# Autodesk Inventor assembly: LINEAR_INTAKE_ASSY
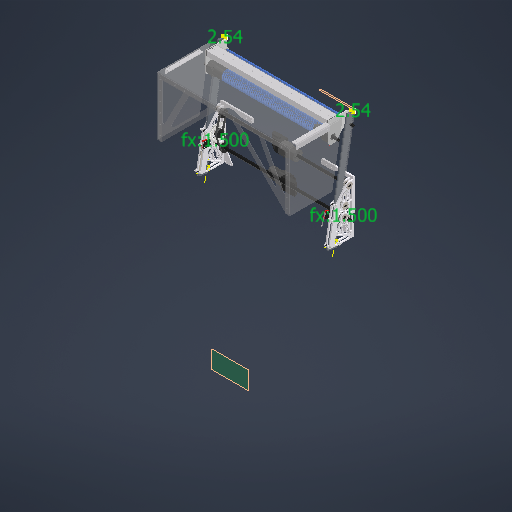
[picture p0: Inventor's stored thumbnail of the model, 512x512]
Saved by Autodesk Inventor 2026.2 (Build 302298010, 298A)
## iProperties
Created: 2026-04-01
Part Number: LINEAR_INTAKE_ASSY
Document SubType Name: Assembly
Designer: 4aida
Author: 4aida
## Documents named in this file (36)
- C:\Users\4aida\OneDrive\Documents\GitHub\2026-Robot-Mechanical\LINEAR_INTAKE\LINEAR_INTAKE_ASSY.iam
- C:\Users\4aida\OneDrive\Documents\GitHub\2026-Robot-Mechanical\LINEAR_INTAKE\0.5_Jack_Shaft.ipt
- C:\Users\4aida\OneDrive\Documents\GitHub\2026-Robot-Mechanical\#1_CAD Library\Electronics\CONTROLS,SPARK_FLEX.ipt
- C:\Users\4aida\OneDrive\Documents\GitHub\2026-Robot-Mechanical\#1_CAD Library\Motors\MOTOR,REV,NEO,VORTEX.ipt
- C:\Users\4aida\OneDrive\Documents\GitHub\2026-Robot-Mechanical\LINEAR_INTAKE\RACK_LINEARINTAKE.ipt
- C:\Users\4aida\OneDrive\Documents\GitHub\2026-Robot-Mechanical\LINEAR_INTAKE\10DP_Pinion Gear.iam
- C:\Users\4aida\OneDrive\Documents\GitHub\2026-Robot-Mechanical\#1_CAD Library\Power Transmission\Bearings\PURCHASED,HEX_BEARING.ipt
- C:\Users\4aida\OneDrive\Documents\GitHub\2026-Robot-Mechanical\LINEAR_INTAKE\INTAKE_OUTSIDE_PLATE.ipt
- C:\Users\4aida\OneDrive\Documents\GitHub\2026-Robot-Mechanical\LINEAR_INTAKE\RACK_GUIDES.ipt
- C:\Users\4aida\OneDrive\Documents\GitHub\2026-Robot-Mechanical\LINEAR_INTAKE\CAST,2inOD,ROLLER.ipt
- C:\Users\4aida\OneDrive\Documents\GitHub\2026-Robot-Mechanical\LINEAR_INTAKE\10dp_Ratio_Gears_INTAKE.iam
- C:\Users\4aida\OneDrive\Documents\GitHub\2026-Robot-Mechanical\LINEAR_INTAKE\INTAKE_EXT_PULLYS.ipt
- C:\Users\4aida\OneDrive\Documents\GitHub\2026-Robot-Mechanical\LINEAR_INTAKE\55t_Belt.ipt
- C:\Users\4aida\OneDrive\Documents\GitHub\2026-Robot-Mechanical\LINEAR_INTAKE\12mm_OD_BEARING.ipt
- C:\Users\4aida\OneDrive\Documents\GitHub\2026-Robot-Mechanical\LINEAR_INTAKE\fastenal_1140891.ipt
- C:\Users\4aida\OneDrive\Documents\GitHub\2026-Robot-Mechanical\LINEAR_INTAKE\SINGLE_BEARING_SPACER.ipt
- C:\Users\4aida\OneDrive\Documents\GitHub\2026-Robot-Mechanical\LINEAR_INTAKE\double_BEARING_SPACER.ipt
- C:\Users\4aida\OneDrive\Documents\GitHub\2026-Robot-Mechanical\LINEAR_INTAKE\INTAKE_SWERVE_MOUNT.ipt
- C:\Users\4aida\OneDrive\Documents\GitHub\2026-Robot-Mechanical\LINEAR_INTAKE\MOUTER_MOUNT_INTAKE.ipt
- C:\Users\4aida\OneDrive\Documents\GitHub\2026-Robot-Mechanical\LINEAR_INTAKE\INTAKE_INSIDE_PLATE.ipt
- C:\Users\4aida\OneDrive\Documents\GitHub\2026-Robot-Mechanical\LINEAR_INTAKE\INTAKE_BACK_MOUNT_PLATE.ipt
- C:\Users\4aida\OneDrive\Documents\GitHub\2026-Robot-Mechanical\LINEAR_INTAKE\PULLY_HEX_SHAFT_INTAKE.ipt
- C:\Users\4aida\OneDrive\Documents\GitHub\2026-Robot-Mechanical\LINEAR_INTAKE\PINION_SHAFT_INTAKE.ipt
- C:\Users\4aida\OneDrive\Documents\GitHub\2026-Robot-Mechanical\LINEAR_INTAKE\TETHLON_TAPE.ipt
- C:\Users\4aida\OneDrive\Documents\GitHub\2026-Robot-Mechanical\LINEAR_INTAKE\PINION_SPACER_INTAKE.ipt
- C:\Users\4aida\OneDrive\Documents\GitHub\2026-Robot-Mechanical\LINEAR_INTAKE\PULLY_SPACER_INTAKE.ipt
- C:\Users\4aida\OneDrive\Documents\GitHub\2026-Robot-Mechanical\LINEAR_INTAKE\1.25IN Roller.iam
- C:\Users\4aida\OneDrive\Documents\GitHub\2026-Robot-Mechanical\LINEAR_INTAKE\CRASH_BAR_INTAKE.ipt
- C:\Users\4aida\OneDrive\Documents\GitHub\2026-Robot-Mechanical\LINEAR_INTAKE\TUBE_PLUGS.ipt
- C:\Users\4aida\OneDrive\Documents\GitHub\2026-Robot-Mechanical\#1_CAD Library\Electronics\CONTROLS,LIMIT_SWITCH,VEX.iam
- C:\Users\4aida\OneDrive\Documents\GitHub\2026-Robot-Mechanical\LINEAR_INTAKE\INSIDE_INTAKE_PLATE.ipt
- C:\Users\4aida\OneDrive\Documents\GitHub\2026-Robot-Mechanical\LINEAR_INTAKE\FRONT_INTAKE_LEXAN.ipt
- C:\Users\4aida\OneDrive\Documents\GitHub\2026-Robot-Mechanical\LINEAR_INTAKE\SIDE_INTAKE_LEXAN.ipt
- C:\Users\4aida\OneDrive\Documents\GitHub\2026-Robot-Mechanical\LINEAR_INTAKE\SIDE_INTAKE_LEXAN_MIR.ipt
- C:\Users\4aida\OneDrive\Documents\GitHub\2026-Robot-Mechanical\LINEAR_INTAKE\TOP_INTAKE_LEXAN.ipt
- C:\Users\4aida\OneDrive\Documents\GitHub\2026-Robot-Mechanical\LINEAR_INTAKE\LEXAN_CORNER_MOUNT.ipt
## Components (130 placed, 35 different names)
1. 0.5_Jack_Shaft:1 — Flush:61
2. CONTROLS,SPARK_FLEX:1 — Mate:104, Angle:1, Mate:132, Mate:134
3. MOTOR,REV,NEO,VORTEX:1 — Mate:133
4. RACK_LINEARINTAKE:1 — Mate:149, Mate:230
5. 10DP_Pinion Gear:1 [sub-assembly] — Mate:19, Mate:201
6. PURCHASED,HEX_BEARING:1
7. PURCHASED,HEX_BEARING:2 — Mate:151, Flush:53, Flush:54
8. INTAKE_OUTSIDE_PLATE:1 — Mate:66, Mate:67, Insert:3, Mate:121, Mate:122, Mate:123, Mate:124, Mate:125, Mate:126, Mate:128, Mate:129, Insert:4, Insert:5, Insert:6, Insert:7, Insert:8, Insert:9, Flush:27, Flush:28, Mate:169, Flush:31, Flush:39, Mate:200, Flush:40
9. INTAKE_OUTSIDE_PLATE:2 — Flush:18, Mate:60, Mate:63, Insert:1, Mate:131, Flush:30, Insert:21, Insert:22, Insert:23, Insert:24, Insert:25, Insert:27, Mate:171, Mate:174, Flush:37, Mate:196, Mate:198, Flush:42, Mate:316, Mate:317
10. RACK_LINEARINTAKE:2
11. 10DP_Pinion Gear:2 [sub-assembly] — Mate:19, Mate:195
12. RACK_GUIDES:1 — Mate:272, Angle:5, Flush:56
13. RACK_GUIDES:4 — Flush:18, Mate:196
14. PURCHASED,HEX_BEARING:3 — Mate:60, Mate:63, Mate:194, Mate:195, Mate:203, Mate:204
15. PURCHASED,HEX_BEARING:4 — Mate:106, Mate:177, Mate:178, Mate:192
16. PURCHASED,HEX_BEARING:5 — Mate:96, Mate:154, Mate:157
17. PURCHASED,HEX_BEARING:6 — Mate:66, Mate:67, Mate:189, Flush:34, Mate:190, Mate:202
18. PURCHASED,HEX_BEARING:7 — Mate:107, Mate:115, Mate:176, Mate:179, Mate:180, Mate:185
19. PURCHASED,HEX_BEARING:8 — Mate:113, Mate:173, Mate:175, Mate:205, Mate:206
20. PURCHASED,HEX_BEARING:9 — Mate:152, Mate:153, Mate:207
21. PURCHASED,HEX_BEARING:10 — Insert:1, Mate:184
22. PURCHASED,HEX_BEARING:11 — Mate:94, Mate:95, Mate:155, Mate:156
23. PURCHASED,HEX_BEARING:12 — Insert:3, Mate:188
24. 55t_Belt:1 — Mate:110, Mate:111, Mate:112, Mate:182, Mate:306
25. 55t_Belt:2 — Mate:99, Mate:100, Mate:101, Mate:102, Mate:158, Mate:293
26. 10dp_Ratio_Gears_INTAKE:3 [sub-assembly] — Mate:94, Mate:95, Mate:96, Mate:97, Mate:98, Mate:154, Mate:191
27. INTAKE_EXT_PULLYS:5 — Mate:97, Mate:98, Mate:99, Mate:100, Flush:33, Mate:186, Mate:187
28. INTAKE_EXT_PULLYS:6 — Mate:101, Mate:102, Mate:208
29. 10dp_Ratio_Gears_INTAKE:4 [sub-assembly] — Mate:106, Mate:107, Mate:108, Mate:109, Mate:110, Flush:35, Mate:193
30. INTAKE_EXT_PULLYS:7 — Mate:108, Mate:109, Mate:111, Flush:26, Mate:115, Flush:32, Mate:183
31. INTAKE_EXT_PULLYS:9 — Mate:112, Flush:26, Mate:113
32. 12mm_OD_BEARING:1 — Mate:121, Mate:124, Insert:13
33. 12mm_OD_BEARING:2 — Mate:119, Mate:120
34. 12mm_OD_BEARING:3 — Mate:125, Insert:11
35. 12mm_OD_BEARING:4 — Mate:122, Mate:123, Insert:15
36. 12mm_OD_BEARING:5 — Mate:119, Mate:120, Insert:10
37. 12mm_OD_BEARING:6 — Mate:126, Insert:12
38. 12mm_OD_BEARING:12 — Mate:128, Mate:129, Insert:14
39. fastenal_1140891:1 — Insert:4
40. fastenal_1140891:2 — Insert:5
41. fastenal_1140891:3 — Insert:8
42. fastenal_1140891:4 — Insert:9
43. fastenal_1140891:5 — Insert:7
44. fastenal_1140891:6 — Insert:6
45. SINGLE_BEARING_SPACER:3 — Insert:10
46. double_BEARING_SPACER:1 — Insert:11
47. double_BEARING_SPACER:2 — Insert:15
48. double_BEARING_SPACER:3 — Insert:12
49. double_BEARING_SPACER:4 — Insert:13
50. double_BEARING_SPACER:5 — Insert:14
51. INTAKE_SWERVE_MOUNT:1 — Flush:27, Flush:28, Flush:29, Mate:150
52. INTAKE_SWERVE_MOUNT:2 — Mate:131, Flush:29, Flush:30, Mate:172, Mate:181, Flush:48
53. MOUTER_MOUNT_INTAKE:1 — Mate:132, Mate:133, Mate:134
54. 12mm_OD_BEARING:13 — Mate:135, Mate:136
55. fastenal_1140891:7 — Mate:135, Mate:136, Insert:24
56. double_BEARING_SPACER:6
57. 12mm_OD_BEARING:14
58. fastenal_1140891:8 — Insert:25
59. double_BEARING_SPACER:7
60. 12mm_OD_BEARING:15
61. fastenal_1140891:9 — Insert:23
62. double_BEARING_SPACER:8
63. 12mm_OD_BEARING:16
64. fastenal_1140891:10 — Insert:21
65. double_BEARING_SPACER:9
66. 12mm_OD_BEARING:17
67. fastenal_1140891:11 — Insert:22
68. double_BEARING_SPACER:10
69. 12mm_OD_BEARING:18
70. 12mm_OD_BEARING:19 — Mate:147
71. fastenal_1140891:12 — Mate:147, Mate:148, Insert:27
72. SINGLE_BEARING_SPACER:4 — Mate:148
73. INTAKE_INSIDE_PLATE:1 — Mate:149, Mate:150, Mate:151, Mate:152, Mate:153, Mate:155, Mate:156, Mate:157, Mate:158, Mate:168, Flush:38, Mate:199, Flush:41, Mate:289, Mate:290, Mate:291, Mate:292, Mate:300
74. INTAKE_BACK_MOUNT_PLATE:1 — Mate:168, Mate:169, Flush:31
75. INTAKE_BACK_MOUNT_PLATE:2 — Mate:171, Mate:315, Mate:316, Mate:317
76. INTAKE_INSIDE_PLATE:3 — Mate:172, Mate:173, Mate:174, Mate:175, Mate:176, Mate:177, Mate:178, Mate:179, Mate:180, Mate:181, Flush:36, Mate:197, Flush:43, Mate:286, Mate:287, Mate:288, Insert:28, Angle:6
77. PULLY_HEX_SHAFT_INTAKE:1 — Mate:182, Flush:32, Mate:183, Mate:184, Mate:185
78. PULLY_HEX_SHAFT_INTAKE:2 — Flush:33, Mate:186, Mate:187, Mate:188
79. PINION_SHAFT_INTAKE:1 — Mate:189, Flush:34, Mate:190, Mate:191
80. PINION_SHAFT_INTAKE:2 — Mate:192, Flush:35, Mate:193, Mate:194
81. TETHLON_TAPE:1 — Flush:36, Mate:197, Flush:43
82. TETHLON_TAPE:2 — Flush:38, Mate:198, Flush:42
83. TETHLON_TAPE:3 — Flush:37, Mate:200, Flush:40
84. TETHLON_TAPE:4 — Flush:39, Mate:199, Flush:41
85. PINION_SPACER_INTAKE:1 — Mate:203, Mate:204
86. PINION_SPACER_INTAKE:2 — Mate:201, Mate:202
87. PULLY_SPACER_INTAKE:1 — Mate:205, Mate:206
88. PULLY_SPACER_INTAKE:2 — Mate:207, Mate:208
89. CRASH_BAR_INTAKE:1 — Mate:220, Mate:224, Mate:225, Mate:226, Mate:227, Mate:228, Mate:229, Mate:230, Angle:2, Mate:274, Flush:55
90. TUBE_PLUGS:1 — Mate:227, Mate:228, Mate:229, Mate:235, Mate:236, Mate:263
91. TUBE_PLUGS:2 — Mate:224, Mate:225, Mate:226, Mate:231, Mate:232, Mate:233
92. INSIDE_INTAKE_PLATE:1 — Mate:231, Mate:232, Mate:233, Mate:242, Mate:243, Mate:244, Mate:249, Mate:250, Angle:4
93. 1.25IN Roller:6 [sub-assembly] — Mate:242, Mate:245, Mate:253, Mate:254, Flush:49
94. INSIDE_INTAKE_PLATE:2 — Mate:235, Mate:236, Mate:240, Mate:241, Angle:3, Mate:262, Mate:263
95. CONTROLS,SPARK_FLEX:4 — Mate:240, Angle:3
96. MOTOR,REV,NEO,VORTEX:4 — Mate:241
97. PURCHASED,HEX_BEARING:14 — Mate:243, Mate:244, Mate:245, Mate:271, Mate:273
98. CAST,2inOD,ROLLER:9 — Mate:251, Mate:252, Mate:264, Mate:267
99. CONTROLS,SPARK_FLEX:5 — Mate:249, Angle:4, Mate:270
100. MOTOR,REV,NEO,VORTEX:5 — Mate:250, Mate:251, Mate:252
101. 1.25IN Roller:7 [sub-assembly] — Mate:253, Mate:254, Mate:255, Mate:256, Flush:49, Flush:50, Flush:51
102. 1.25IN Roller:8 [sub-assembly] — Mate:255, Mate:256, Flush:50, Mate:257, Mate:258, Flush:51
103. 1.25IN Roller:9 [sub-assembly] — Mate:257, Mate:258, Mate:259, Mate:260, Flush:52
104. 1.25IN Roller:10 [sub-assembly] — Mate:259, Mate:260, Flush:52, Mate:261
105. PURCHASED,HEX_BEARING:15 — Mate:261, Mate:262
106. CAST,2inOD,ROLLER:10 — Mate:264, Mate:265, Mate:267, Mate:268
107. CAST,2inOD,ROLLER:11 — Mate:265, Mate:266, Mate:268, Mate:269
108. CAST,2inOD,ROLLER:12 — Mate:266, Mate:269
109. 0.5_Jack_Shaft:2 — Flush:53, Mate:270
110. 0.5_Jack_Shaft:3 — Flush:54, Mate:271
111. FRONT_INTAKE_LEXAN:2 — Mate:274, Flush:55, Flush:56, Mate:275, Mate:276, Flush:57, Mate:277, Flush:58, Mate:278, Flush:60, Mate:280, Mate:282, Mate:285
112. SIDE_INTAKE_LEXAN:1 — Mate:275, Mate:276, Flush:57, Mate:281
113. SIDE_INTAKE_LEXAN_MIR:1 — Mate:277, Flush:58, Mate:278, Mate:279, Flush:59, Mate:283, Mate:284
114. TOP_INTAKE_LEXAN:1 — Mate:279, Flush:59, Flush:60
115. LEXAN_CORNER_MOUNT:1 — Mate:280, Mate:281, Mate:285
116. LEXAN_CORNER_MOUNT:2 — Mate:282, Mate:283, Mate:284
117. CONTROLS,LIMIT_SWITCH,VEX:2 [sub-assembly] — Mate:286, Mate:287, Mate:288
118. CONTROLS,LIMIT_SWITCH,VEX:3 [sub-assembly] — Mate:289, Mate:290, Mate:291
119. PURCHASED,HEX_BEARING:16 — Mate:292, Mate:294, Mate:299, Mate:300
120. 55t_Belt:3 — Mate:293, Mate:294, Mate:295, Mate:296
121. INTAKE_EXT_PULLYS:10 — Mate:295, Mate:296, Mate:297, Mate:298, Mate:301
122. PULLY_SPACER_INTAKE:3 — Mate:297, Mate:298, Mate:299
123. 0.5_Jack_Shaft:4 — Mate:301, Flush:61
124. PURCHASED,HEX_BEARING:17 — Insert:28
125. INTAKE_EXT_PULLYS:11 — Mate:305, Mate:307, Mate:308
126. PULLY_SPACER_INTAKE:4 — Mate:305
127. 55t_Belt:4 — Mate:306, Mate:307, Mate:308
128. CONTROLS,SPARK_FLEX:6
129. MOTOR,REV,NEO,VORTEX:6
130. MOUTER_MOUNT_INTAKE:2 — Mate:315, Angle:6
## Relationships (289: Mate 212, Flush 44, Insert 27, Angle 6)
- [Mate]: CONTROLS,SPARK_FLEX:1 ↔ MOTOR,REV,NEO,VORTEX:1
- [Mate]: CONTROLS,SPARK_FLEX:1 ↔ MOTOR,REV,NEO,VORTEX:1
- [Mate]: CONTROLS,SPARK_FLEX:1 ↔ MOTOR,REV,NEO,VORTEX:1
- [Mate]: 0.5_Jack_Shaft:1 ↔ CONTROLS,SPARK_FLEX:1
- [Mate]: 0.5_Jack_Shaft:1 ↔ MOTOR,REV,NEO,VORTEX:1
- [Flush]: RACK_LINEARINTAKE:1 ↔ 10DP_Pinion Gear:1
- [Flush]: 0.5_Jack_Shaft:1 ↔ PURCHASED,HEX_BEARING:2
- [Flush]: 0.5_Jack_Shaft:1 ↔ PURCHASED,HEX_BEARING:1
- [Mate]: 0.5_Jack_Shaft:1 ↔ PURCHASED,HEX_BEARING:1
- [Mate]: 0.5_Jack_Shaft:1 ↔ PURCHASED,HEX_BEARING:2
- [Mate]: 0.5_Jack_Shaft:1 ↔ PURCHASED,HEX_BEARING:2
- [Mate]: 0.5_Jack_Shaft:1 ↔ PURCHASED,HEX_BEARING:1
- [Mate]: PURCHASED,HEX_BEARING:2 ↔ INTAKE_OUTSIDE_PLATE:1
- [Mate]: PURCHASED,HEX_BEARING:2 ↔ INTAKE_OUTSIDE_PLATE:1
- [Flush] (6 mm): RACK_LINEARINTAKE:1 ↔ INTAKE_OUTSIDE_PLATE:1
- [Mate] (5.2705 mm): RACK_LINEARINTAKE:1 ↔ INTAKE_OUTSIDE_PLATE:1
- [Mate]: PURCHASED,HEX_BEARING:1 ↔ INTAKE_OUTSIDE_PLATE:2
- [Mate]: PURCHASED,HEX_BEARING:1 ↔ INTAKE_OUTSIDE_PLATE:2
- [Flush]: RACK_LINEARINTAKE:2 ↔ 10DP_Pinion Gear:2
- [Flush]: RACK_LINEARINTAKE:1 ↔ RACK_LINEARINTAKE:2
- [Flush]: RACK_LINEARINTAKE:1 ↔ RACK_LINEARINTAKE:2
- Mate:19: 10DP_Pinion Gear:1 ↔ 10DP_Pinion Gear:2
- [Mate]: RACK_LINEARINTAKE:1 ↔ RACK_GUIDES:1
- [Mate]: RACK_LINEARINTAKE:2 ↔ RACK_GUIDES:4
- [Flush]: RACK_LINEARINTAKE:2 ↔ RACK_GUIDES:4
- [Flush]: RACK_LINEARINTAKE:2 ↔ RACK_GUIDES:4
- [Flush]: RACK_LINEARINTAKE:1 ↔ RACK_GUIDES:1
- [Flush]: RACK_LINEARINTAKE:1 ↔ RACK_GUIDES:1
- Flush:18: INTAKE_OUTSIDE_PLATE:2 ↔ RACK_GUIDES:4
- Mate:60: INTAKE_OUTSIDE_PLATE:2 ↔ PURCHASED,HEX_BEARING:3
- Mate:63: INTAKE_OUTSIDE_PLATE:2 ↔ PURCHASED,HEX_BEARING:3
- Mate:66: INTAKE_OUTSIDE_PLATE:1 ↔ PURCHASED,HEX_BEARING:6
- Mate:67: INTAKE_OUTSIDE_PLATE:1 ↔ PURCHASED,HEX_BEARING:6
- Insert:1: INTAKE_OUTSIDE_PLATE:2 ↔ PURCHASED,HEX_BEARING:10
- Insert:3: INTAKE_OUTSIDE_PLATE:1 ↔ PURCHASED,HEX_BEARING:12
- Mate:94: PURCHASED,HEX_BEARING:11 ↔ 10dp_Ratio_Gears_INTAKE:3
- Mate:95: PURCHASED,HEX_BEARING:11 ↔ 10dp_Ratio_Gears_INTAKE:3
- Mate:96: PURCHASED,HEX_BEARING:5 ↔ 10dp_Ratio_Gears_INTAKE:3
- Mate:97: 10dp_Ratio_Gears_INTAKE:3 ↔ INTAKE_EXT_PULLYS:5
- Mate:98: 10dp_Ratio_Gears_INTAKE:3 ↔ INTAKE_EXT_PULLYS:5
- Mate:99: 55t_Belt:2 ↔ INTAKE_EXT_PULLYS:5
- Mate:100: 55t_Belt:2 ↔ INTAKE_EXT_PULLYS:5
- Mate:101: 55t_Belt:2 ↔ INTAKE_EXT_PULLYS:6
- Mate:102: 55t_Belt:2 ↔ INTAKE_EXT_PULLYS:6
- Mate:104: CONTROLS,SPARK_FLEX:1
- Mate:106: PURCHASED,HEX_BEARING:4 ↔ 10dp_Ratio_Gears_INTAKE:4
- Mate:107: PURCHASED,HEX_BEARING:7 ↔ 10dp_Ratio_Gears_INTAKE:4
- Mate:108: 10dp_Ratio_Gears_INTAKE:4 ↔ INTAKE_EXT_PULLYS:7
- Mate:109: 10dp_Ratio_Gears_INTAKE:4 ↔ INTAKE_EXT_PULLYS:7
- Mate:110: 55t_Belt:1 ↔ 10dp_Ratio_Gears_INTAKE:4
- Mate:111: 55t_Belt:1 ↔ INTAKE_EXT_PULLYS:7
- Mate:112: 55t_Belt:1 ↔ INTAKE_EXT_PULLYS:9
- Flush:26: INTAKE_EXT_PULLYS:7 ↔ INTAKE_EXT_PULLYS:9
- Mate:113: PURCHASED,HEX_BEARING:8 ↔ INTAKE_EXT_PULLYS:9
- Mate:115: PURCHASED,HEX_BEARING:7 ↔ INTAKE_EXT_PULLYS:7
- Angle:1 (0 deg): CONTROLS,SPARK_FLEX:1
- Mate:119: 12mm_OD_BEARING:2 ↔ 12mm_OD_BEARING:5
- Mate:120: 12mm_OD_BEARING:2 ↔ 12mm_OD_BEARING:5
- Mate:121: INTAKE_OUTSIDE_PLATE:1 ↔ 12mm_OD_BEARING:1
- Mate:122: INTAKE_OUTSIDE_PLATE:1 ↔ 12mm_OD_BEARING:4
- Mate:123: INTAKE_OUTSIDE_PLATE:1 ↔ 12mm_OD_BEARING:4
- Mate:124: INTAKE_OUTSIDE_PLATE:1 ↔ 12mm_OD_BEARING:1
- Mate:125: INTAKE_OUTSIDE_PLATE:1 ↔ 12mm_OD_BEARING:3
- Mate:126: INTAKE_OUTSIDE_PLATE:1 ↔ 12mm_OD_BEARING:6
- Mate:128: INTAKE_OUTSIDE_PLATE:1 ↔ 12mm_OD_BEARING:12
- Mate:129: INTAKE_OUTSIDE_PLATE:1 ↔ 12mm_OD_BEARING:12
- Insert:4: INTAKE_OUTSIDE_PLATE:1 ↔ fastenal_1140891:1
- Insert:5: INTAKE_OUTSIDE_PLATE:1 ↔ fastenal_1140891:2
- Insert:6: INTAKE_OUTSIDE_PLATE:1 ↔ fastenal_1140891:6
- Insert:7: INTAKE_OUTSIDE_PLATE:1 ↔ fastenal_1140891:5
- Insert:8: INTAKE_OUTSIDE_PLATE:1 ↔ fastenal_1140891:3
- Insert:9: INTAKE_OUTSIDE_PLATE:1 ↔ fastenal_1140891:4
- Insert:10: 12mm_OD_BEARING:5 ↔ SINGLE_BEARING_SPACER:3
- Insert:11: 12mm_OD_BEARING:3 ↔ double_BEARING_SPACER:1
- Insert:12: 12mm_OD_BEARING:6 ↔ double_BEARING_SPACER:3
- Insert:13: 12mm_OD_BEARING:1 ↔ double_BEARING_SPACER:4
- Insert:14: 12mm_OD_BEARING:12 ↔ double_BEARING_SPACER:5
- Insert:15: 12mm_OD_BEARING:4 ↔ double_BEARING_SPACER:2
- Flush:27: INTAKE_OUTSIDE_PLATE:1 ↔ INTAKE_SWERVE_MOUNT:1
- Flush:28 (-12.2199 mm): INTAKE_OUTSIDE_PLATE:1 ↔ INTAKE_SWERVE_MOUNT:1
- Mate:131: INTAKE_OUTSIDE_PLATE:2 ↔ INTAKE_SWERVE_MOUNT:2
- Flush:29: INTAKE_SWERVE_MOUNT:1 ↔ INTAKE_SWERVE_MOUNT:2
- Flush:30: INTAKE_OUTSIDE_PLATE:2 ↔ INTAKE_SWERVE_MOUNT:2
- Mate:132: CONTROLS,SPARK_FLEX:1 ↔ MOUTER_MOUNT_INTAKE:1
- Mate:133: MOTOR,REV,NEO,VORTEX:1 ↔ MOUTER_MOUNT_INTAKE:1
- Mate:134: CONTROLS,SPARK_FLEX:1 ↔ MOUTER_MOUNT_INTAKE:1
- [Insert]: 12mm_OD_BEARING:13 ↔ double_BEARING_SPACER:6
- Mate:135 (6.35 mm): 12mm_OD_BEARING:13 ↔ fastenal_1140891:7
- Mate:136: 12mm_OD_BEARING:13 ↔ fastenal_1140891:7
- [Insert]: 12mm_OD_BEARING:14 ↔ double_BEARING_SPACER:7
- [Mate] (6.35 mm): 12mm_OD_BEARING:14 ↔ fastenal_1140891:8
- [Mate]: 12mm_OD_BEARING:14 ↔ fastenal_1140891:8
- [Insert]: 12mm_OD_BEARING:15 ↔ double_BEARING_SPACER:8
- [Mate] (6.35 mm): 12mm_OD_BEARING:15 ↔ fastenal_1140891:9
- [Mate]: 12mm_OD_BEARING:15 ↔ fastenal_1140891:9
- [Insert]: 12mm_OD_BEARING:16 ↔ double_BEARING_SPACER:9
- [Mate] (6.35 mm): 12mm_OD_BEARING:16 ↔ fastenal_1140891:10
- [Mate]: 12mm_OD_BEARING:16 ↔ fastenal_1140891:10
- [Insert]: 12mm_OD_BEARING:17 ↔ double_BEARING_SPACER:10
- [Mate] (6.35 mm): 12mm_OD_BEARING:17 ↔ fastenal_1140891:11
- [Mate]: 12mm_OD_BEARING:17 ↔ fastenal_1140891:11
- Insert:21: INTAKE_OUTSIDE_PLATE:2 ↔ fastenal_1140891:10
- Insert:22: INTAKE_OUTSIDE_PLATE:2 ↔ fastenal_1140891:11
- Insert:23: INTAKE_OUTSIDE_PLATE:2 ↔ fastenal_1140891:9
- Insert:24: INTAKE_OUTSIDE_PLATE:2 ↔ fastenal_1140891:7
- Insert:25: INTAKE_OUTSIDE_PLATE:2 ↔ fastenal_1140891:8
- [Mate]: 12mm_OD_BEARING:18 ↔ 12mm_OD_BEARING:19
- [Mate]: 12mm_OD_BEARING:18 ↔ 12mm_OD_BEARING:19
- [Insert]: 12mm_OD_BEARING:19 ↔ SINGLE_BEARING_SPACER:4
- Mate:147: 12mm_OD_BEARING:19 ↔ fastenal_1140891:12
- Mate:148 (6.35 mm): fastenal_1140891:12 ↔ SINGLE_BEARING_SPACER:4
- Insert:27: INTAKE_OUTSIDE_PLATE:2 ↔ fastenal_1140891:12
- Mate:149 (0.508 mm): RACK_LINEARINTAKE:1 ↔ INTAKE_INSIDE_PLATE:1
- Mate:150: INTAKE_SWERVE_MOUNT:1 ↔ INTAKE_INSIDE_PLATE:1
- Mate:151: PURCHASED,HEX_BEARING:2 ↔ INTAKE_INSIDE_PLATE:1
- Mate:152: PURCHASED,HEX_BEARING:9 ↔ INTAKE_INSIDE_PLATE:1
- Mate:153: PURCHASED,HEX_BEARING:9 ↔ INTAKE_INSIDE_PLATE:1
- Mate:154: PURCHASED,HEX_BEARING:5 ↔ 10dp_Ratio_Gears_INTAKE:3
- Mate:155: PURCHASED,HEX_BEARING:11 ↔ INTAKE_INSIDE_PLATE:1
- Mate:156: PURCHASED,HEX_BEARING:11 ↔ INTAKE_INSIDE_PLATE:1
- Mate:157: PURCHASED,HEX_BEARING:5 ↔ INTAKE_INSIDE_PLATE:1
- Mate:158: 55t_Belt:2 ↔ INTAKE_INSIDE_PLATE:1
- Mate:168: INTAKE_INSIDE_PLATE:1 ↔ INTAKE_BACK_MOUNT_PLATE:1
- Mate:169: INTAKE_OUTSIDE_PLATE:1 ↔ INTAKE_BACK_MOUNT_PLATE:1
- Flush:31: INTAKE_OUTSIDE_PLATE:1 ↔ INTAKE_BACK_MOUNT_PLATE:1
- Mate:171: INTAKE_OUTSIDE_PLATE:2 ↔ INTAKE_BACK_MOUNT_PLATE:2
- Mate:172: INTAKE_SWERVE_MOUNT:2 ↔ INTAKE_INSIDE_PLATE:3
- Mate:173: PURCHASED,HEX_BEARING:8 ↔ INTAKE_INSIDE_PLATE:3
- Mate:174: INTAKE_OUTSIDE_PLATE:2 ↔ INTAKE_INSIDE_PLATE:3
- Mate:175: PURCHASED,HEX_BEARING:8 ↔ INTAKE_INSIDE_PLATE:3
- Mate:176: PURCHASED,HEX_BEARING:7 ↔ INTAKE_INSIDE_PLATE:3
- Mate:177: PURCHASED,HEX_BEARING:4 ↔ INTAKE_INSIDE_PLATE:3
- Mate:178: PURCHASED,HEX_BEARING:4 ↔ INTAKE_INSIDE_PLATE:3
- Mate:179: PURCHASED,HEX_BEARING:7 ↔ INTAKE_INSIDE_PLATE:3
- Mate:180: PURCHASED,HEX_BEARING:7 ↔ INTAKE_INSIDE_PLATE:3
- Mate:181: INTAKE_SWERVE_MOUNT:2 ↔ INTAKE_INSIDE_PLATE:3
- Mate:182: 55t_Belt:1 ↔ PULLY_HEX_SHAFT_INTAKE:1
- Flush:32: INTAKE_EXT_PULLYS:7 ↔ PULLY_HEX_SHAFT_INTAKE:1
- Mate:183: INTAKE_EXT_PULLYS:7 ↔ PULLY_HEX_SHAFT_INTAKE:1
- Mate:184: PURCHASED,HEX_BEARING:10 ↔ PULLY_HEX_SHAFT_INTAKE:1
- Mate:185: PURCHASED,HEX_BEARING:7 ↔ PULLY_HEX_SHAFT_INTAKE:1
- Flush:33: INTAKE_EXT_PULLYS:5 ↔ PULLY_HEX_SHAFT_INTAKE:2
- Mate:186: INTAKE_EXT_PULLYS:5 ↔ PULLY_HEX_SHAFT_INTAKE:2
- Mate:187: INTAKE_EXT_PULLYS:5 ↔ PULLY_HEX_SHAFT_INTAKE:2
- Mate:188: PURCHASED,HEX_BEARING:12 ↔ PULLY_HEX_SHAFT_INTAKE:2
- Mate:189: PURCHASED,HEX_BEARING:6 ↔ PINION_SHAFT_INTAKE:1
- Flush:34: PURCHASED,HEX_BEARING:6 ↔ PINION_SHAFT_INTAKE:1
- Mate:190: PURCHASED,HEX_BEARING:6 ↔ PINION_SHAFT_INTAKE:1
- Mate:191: 10dp_Ratio_Gears_INTAKE:3 ↔ PINION_SHAFT_INTAKE:1
- Mate:192: PURCHASED,HEX_BEARING:4 ↔ PINION_SHAFT_INTAKE:2
- Flush:35: 10dp_Ratio_Gears_INTAKE:4 ↔ PINION_SHAFT_INTAKE:2
- Mate:193: 10dp_Ratio_Gears_INTAKE:4 ↔ PINION_SHAFT_INTAKE:2
- Mate:194: PURCHASED,HEX_BEARING:3 ↔ PINION_SHAFT_INTAKE:2
- Flush:36: INTAKE_INSIDE_PLATE:3 ↔ TETHLON_TAPE:1
- Flush:37: INTAKE_OUTSIDE_PLATE:2 ↔ TETHLON_TAPE:3
- Flush:38: INTAKE_INSIDE_PLATE:1 ↔ TETHLON_TAPE:2
- Flush:39: INTAKE_OUTSIDE_PLATE:1 ↔ TETHLON_TAPE:4
- Mate:195: 10DP_Pinion Gear:2 ↔ PURCHASED,HEX_BEARING:3
- Mate:196 (0.508 mm): INTAKE_OUTSIDE_PLATE:2 ↔ RACK_GUIDES:4
- Mate:197: INTAKE_INSIDE_PLATE:3 ↔ TETHLON_TAPE:1
- Mate:198: INTAKE_OUTSIDE_PLATE:2 ↔ TETHLON_TAPE:2
- Mate:199: INTAKE_INSIDE_PLATE:1 ↔ TETHLON_TAPE:4
- Mate:200: INTAKE_OUTSIDE_PLATE:1 ↔ TETHLON_TAPE:3
- Flush:40: INTAKE_OUTSIDE_PLATE:1 ↔ TETHLON_TAPE:3
- Flush:41: INTAKE_INSIDE_PLATE:1 ↔ TETHLON_TAPE:4
- Flush:42: INTAKE_OUTSIDE_PLATE:2 ↔ TETHLON_TAPE:2
- Flush:43: INTAKE_INSIDE_PLATE:3 ↔ TETHLON_TAPE:1
- Mate:201: 10DP_Pinion Gear:1 ↔ PINION_SPACER_INTAKE:2
- Mate:202: PURCHASED,HEX_BEARING:6 ↔ PINION_SPACER_INTAKE:2
- Mate:203: PURCHASED,HEX_BEARING:3 ↔ PINION_SPACER_INTAKE:1
- Mate:204: PURCHASED,HEX_BEARING:3 ↔ PINION_SPACER_INTAKE:1
- Mate:205: PURCHASED,HEX_BEARING:8 ↔ PULLY_SPACER_INTAKE:1
- Mate:206: PURCHASED,HEX_BEARING:8 ↔ PULLY_SPACER_INTAKE:1
- Mate:207: PURCHASED,HEX_BEARING:9 ↔ PULLY_SPACER_INTAKE:2
- Mate:208: INTAKE_EXT_PULLYS:6 ↔ PULLY_SPACER_INTAKE:2
- Flush:48 (304.8 mm): INTAKE_SWERVE_MOUNT:2
- Mate:220: CRASH_BAR_INTAKE:1
- Mate:224: CRASH_BAR_INTAKE:1 ↔ TUBE_PLUGS:2
- Mate:225: CRASH_BAR_INTAKE:1 ↔ TUBE_PLUGS:2
- Mate:226: CRASH_BAR_INTAKE:1 ↔ TUBE_PLUGS:2
- Mate:227: CRASH_BAR_INTAKE:1 ↔ TUBE_PLUGS:1
- Mate:228: CRASH_BAR_INTAKE:1 ↔ TUBE_PLUGS:1
- Mate:229: CRASH_BAR_INTAKE:1 ↔ TUBE_PLUGS:1
- Mate:230: RACK_LINEARINTAKE:1 ↔ CRASH_BAR_INTAKE:1
- Angle:2 (0 deg): CRASH_BAR_INTAKE:1
- Mate:231: TUBE_PLUGS:2 ↔ INSIDE_INTAKE_PLATE:1
- Mate:232: TUBE_PLUGS:2 ↔ INSIDE_INTAKE_PLATE:1
- Mate:233: TUBE_PLUGS:2 ↔ INSIDE_INTAKE_PLATE:1
- Mate:235: TUBE_PLUGS:1 ↔ INSIDE_INTAKE_PLATE:2
- Mate:236: TUBE_PLUGS:1 ↔ INSIDE_INTAKE_PLATE:2
- [Mate]: CONTROLS,SPARK_FLEX:4 ↔ MOTOR,REV,NEO,VORTEX:4
- [Mate]: CONTROLS,SPARK_FLEX:4 ↔ MOTOR,REV,NEO,VORTEX:4
- [Mate]: CONTROLS,SPARK_FLEX:4 ↔ MOTOR,REV,NEO,VORTEX:4
- Mate:240: INSIDE_INTAKE_PLATE:2 ↔ CONTROLS,SPARK_FLEX:4
- Mate:241: INSIDE_INTAKE_PLATE:2 ↔ MOTOR,REV,NEO,VORTEX:4
- Angle:3 (90 deg): INSIDE_INTAKE_PLATE:2 ↔ CONTROLS,SPARK_FLEX:4
- Mate:242: INSIDE_INTAKE_PLATE:1 ↔ 1.25IN Roller:6
- Mate:243: INSIDE_INTAKE_PLATE:1 ↔ PURCHASED,HEX_BEARING:14
- Mate:244: INSIDE_INTAKE_PLATE:1 ↔ PURCHASED,HEX_BEARING:14
- Mate:245: 1.25IN Roller:6 ↔ PURCHASED,HEX_BEARING:14
- [Mate]: CONTROLS,SPARK_FLEX:5 ↔ MOTOR,REV,NEO,VORTEX:5
- [Mate]: CONTROLS,SPARK_FLEX:5 ↔ MOTOR,REV,NEO,VORTEX:5
- [Mate]: CONTROLS,SPARK_FLEX:5 ↔ MOTOR,REV,NEO,VORTEX:5
- Mate:249: INSIDE_INTAKE_PLATE:1 ↔ CONTROLS,SPARK_FLEX:5
- Mate:250: INSIDE_INTAKE_PLATE:1 ↔ MOTOR,REV,NEO,VORTEX:5
- Angle:4 (90 deg): INSIDE_INTAKE_PLATE:1 ↔ CONTROLS,SPARK_FLEX:5
- Mate:251: CAST,2inOD,ROLLER:9 ↔ MOTOR,REV,NEO,VORTEX:5
- Mate:252: CAST,2inOD,ROLLER:9 ↔ MOTOR,REV,NEO,VORTEX:5
- Mate:253: 1.25IN Roller:6 ↔ 1.25IN Roller:7
- Mate:254: 1.25IN Roller:6 ↔ 1.25IN Roller:7
- Mate:255: 1.25IN Roller:7 ↔ 1.25IN Roller:8
- Mate:256: 1.25IN Roller:7 ↔ 1.25IN Roller:8
- Flush:49: 1.25IN Roller:6 ↔ 1.25IN Roller:7
- Flush:50: 1.25IN Roller:7 ↔ 1.25IN Roller:8
- Mate:257: 1.25IN Roller:8 ↔ 1.25IN Roller:9
- Mate:258: 1.25IN Roller:8 ↔ 1.25IN Roller:9
- Flush:51: 1.25IN Roller:7 ↔ 1.25IN Roller:8
- Mate:259: 1.25IN Roller:9 ↔ 1.25IN Roller:10
- Mate:260: 1.25IN Roller:9 ↔ 1.25IN Roller:10
- Flush:52: 1.25IN Roller:9 ↔ 1.25IN Roller:10
- Mate:261: 1.25IN Roller:10 ↔ PURCHASED,HEX_BEARING:15
- Mate:262: INSIDE_INTAKE_PLATE:2 ↔ PURCHASED,HEX_BEARING:15
- Mate:263: TUBE_PLUGS:1 ↔ INSIDE_INTAKE_PLATE:2
- Mate:264: CAST,2inOD,ROLLER:9 ↔ CAST,2inOD,ROLLER:10
- Mate:265: CAST,2inOD,ROLLER:10 ↔ CAST,2inOD,ROLLER:11
- Mate:266: CAST,2inOD,ROLLER:11 ↔ CAST,2inOD,ROLLER:12
- Mate:267: CAST,2inOD,ROLLER:9 ↔ CAST,2inOD,ROLLER:10
- Mate:268: CAST,2inOD,ROLLER:10 ↔ CAST,2inOD,ROLLER:11
- Mate:269: CAST,2inOD,ROLLER:11 ↔ CAST,2inOD,ROLLER:12
- Flush:53: PURCHASED,HEX_BEARING:2 ↔ 0.5_Jack_Shaft:2
- Flush:54: PURCHASED,HEX_BEARING:2 ↔ 0.5_Jack_Shaft:3
- Mate:270: CONTROLS,SPARK_FLEX:5 ↔ 0.5_Jack_Shaft:2
- Mate:271: PURCHASED,HEX_BEARING:14 ↔ 0.5_Jack_Shaft:3
- Mate:272: RACK_GUIDES:1
- Angle:5 (10 deg): RACK_GUIDES:1
- Mate:273 (-17.1381 mm): PURCHASED,HEX_BEARING:14
- Mate:274: CRASH_BAR_INTAKE:1 ↔ FRONT_INTAKE_LEXAN:2
- Flush:55: CRASH_BAR_INTAKE:1 ↔ FRONT_INTAKE_LEXAN:2
- Flush:56 (-3.175 mm): RACK_GUIDES:1 ↔ FRONT_INTAKE_LEXAN:2
- Mate:275: FRONT_INTAKE_LEXAN:2 ↔ SIDE_INTAKE_LEXAN:1
- Mate:276: FRONT_INTAKE_LEXAN:2 ↔ SIDE_INTAKE_LEXAN:1
- Flush:57: FRONT_INTAKE_LEXAN:2 ↔ SIDE_INTAKE_LEXAN:1
- Mate:277: FRONT_INTAKE_LEXAN:2 ↔ SIDE_INTAKE_LEXAN_MIR:1
- Flush:58: FRONT_INTAKE_LEXAN:2 ↔ SIDE_INTAKE_LEXAN_MIR:1
- Mate:278: FRONT_INTAKE_LEXAN:2 ↔ SIDE_INTAKE_LEXAN_MIR:1
- Mate:279: SIDE_INTAKE_LEXAN_MIR:1 ↔ TOP_INTAKE_LEXAN:1
- Flush:59: SIDE_INTAKE_LEXAN_MIR:1 ↔ TOP_INTAKE_LEXAN:1
- Flush:60: FRONT_INTAKE_LEXAN:2 ↔ TOP_INTAKE_LEXAN:1
- Mate:280: FRONT_INTAKE_LEXAN:2 ↔ LEXAN_CORNER_MOUNT:1
- Mate:281: SIDE_INTAKE_LEXAN:1 ↔ LEXAN_CORNER_MOUNT:1
- Mate:282: FRONT_INTAKE_LEXAN:2 ↔ LEXAN_CORNER_MOUNT:2
- Mate:283: SIDE_INTAKE_LEXAN_MIR:1 ↔ LEXAN_CORNER_MOUNT:2
- Mate:284: SIDE_INTAKE_LEXAN_MIR:1 ↔ LEXAN_CORNER_MOUNT:2
- Mate:285: FRONT_INTAKE_LEXAN:2 ↔ LEXAN_CORNER_MOUNT:1
- Mate:286: INTAKE_INSIDE_PLATE:3 ↔ CONTROLS,LIMIT_SWITCH,VEX:2
- Mate:287 (-12.7 mm): INTAKE_INSIDE_PLATE:3 ↔ CONTROLS,LIMIT_SWITCH,VEX:2
- Mate:288: INTAKE_INSIDE_PLATE:3 ↔ CONTROLS,LIMIT_SWITCH,VEX:2
- Mate:289: INTAKE_INSIDE_PLATE:1 ↔ CONTROLS,LIMIT_SWITCH,VEX:3
- Mate:290: INTAKE_INSIDE_PLATE:1 ↔ CONTROLS,LIMIT_SWITCH,VEX:3
- Mate:291: INTAKE_INSIDE_PLATE:1 ↔ CONTROLS,LIMIT_SWITCH,VEX:3
- Mate:292: INTAKE_INSIDE_PLATE:1 ↔ PURCHASED,HEX_BEARING:16
- Mate:293: 55t_Belt:2 ↔ 55t_Belt:3
- Mate:294: PURCHASED,HEX_BEARING:16 ↔ 55t_Belt:3
- Mate:295: 55t_Belt:3 ↔ INTAKE_EXT_PULLYS:10
- Mate:296: 55t_Belt:3 ↔ INTAKE_EXT_PULLYS:10
- Mate:297: INTAKE_EXT_PULLYS:10 ↔ PULLY_SPACER_INTAKE:3
- Mate:298: INTAKE_EXT_PULLYS:10 ↔ PULLY_SPACER_INTAKE:3
- Mate:299: PURCHASED,HEX_BEARING:16 ↔ PULLY_SPACER_INTAKE:3
- Mate:300: INTAKE_INSIDE_PLATE:1 ↔ PURCHASED,HEX_BEARING:16
- Mate:301: INTAKE_EXT_PULLYS:10 ↔ 0.5_Jack_Shaft:4
- Flush:61: 0.5_Jack_Shaft:1 ↔ 0.5_Jack_Shaft:4
- [Mate]: PURCHASED,HEX_BEARING:17 ↔ INTAKE_EXT_PULLYS:11
- [Mate]: PURCHASED,HEX_BEARING:17 ↔ PULLY_SPACER_INTAKE:4
- [Mate]: PURCHASED,HEX_BEARING:17 ↔ PULLY_SPACER_INTAKE:4
- Insert:28: INTAKE_INSIDE_PLATE:3 ↔ PURCHASED,HEX_BEARING:17
- Mate:305: INTAKE_EXT_PULLYS:11 ↔ PULLY_SPACER_INTAKE:4
- Mate:306: 55t_Belt:1 ↔ 55t_Belt:4
- Mate:307: INTAKE_EXT_PULLYS:11 ↔ 55t_Belt:4
- Mate:308: INTAKE_EXT_PULLYS:11 ↔ 55t_Belt:4
- [Mate]: CONTROLS,SPARK_FLEX:6 ↔ MOTOR,REV,NEO,VORTEX:6
- [Mate]: CONTROLS,SPARK_FLEX:6 ↔ MOTOR,REV,NEO,VORTEX:6
- [Mate]: CONTROLS,SPARK_FLEX:6 ↔ MOTOR,REV,NEO,VORTEX:6
- [Mate]: CONTROLS,SPARK_FLEX:6 ↔ MOUTER_MOUNT_INTAKE:2
- [Mate]: MOTOR,REV,NEO,VORTEX:6 ↔ MOUTER_MOUNT_INTAKE:2
- [Mate]: CONTROLS,SPARK_FLEX:6 ↔ MOUTER_MOUNT_INTAKE:2
- Mate:315 (3.175 mm): INTAKE_BACK_MOUNT_PLATE:2 ↔ MOUTER_MOUNT_INTAKE:2
- Mate:316: INTAKE_OUTSIDE_PLATE:2 ↔ INTAKE_BACK_MOUNT_PLATE:2
- Mate:317: INTAKE_OUTSIDE_PLATE:2 ↔ INTAKE_BACK_MOUNT_PLATE:2
- Angle:6 (0 deg): INTAKE_INSIDE_PLATE:3 ↔ MOUTER_MOUNT_INTAKE:2
## Named parameters: d193_d174 = 0 mm, d163_d8 = 0 mm, d164_d9 = 0 mm, d165_d10 = 0 mm, d265_d252 = 0 mm, d268_d265_d252 = 0 mm, d269_d266 = 6.35 mm, d270_d267 = 0 mm, d271_d265_d252 = 0 mm, d272_d266 = 6.35 mm, d273_d267 = 0 mm, d274_d265_d252 = 0 mm, d275_d266 = 6.35 mm, d276_d267 = 0 mm, d277_d265_d252 = 0 mm, d278_d266 = 6.35 mm, d279_d267 = 0 mm, d285_d250 = 0 mm, d286_d229 = 0 mm, d287_d230 = 0 mm, d406_d72_d163_d8 = 0 mm, d407_d73_d164_d9 = 0 mm, d408_d74_d165_d10 = 0 mm, d416_d75_d163_d8 = 0 mm, d417_d76_d164_d9 = 0 mm, d418_d77_d165_d10 = 0 mm, d493_d201 = 0 mm, d494_d361 = 0 mm, d495_d362 = 0 mm, d501_d262 = 0 mm, d502_d263 = 0 mm, d503_d264 = 0 mm, d504_d163_d8 = 0 mm, d505_d164_d9 = 0 mm, d506_d165_d10 = 0 mm
